# Autodesk Inventor assembly: Assembly1
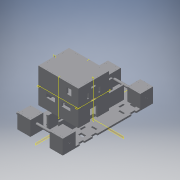
[picture p0: Inventor's stored thumbnail of the model, 180x180]
Saved by Autodesk Inventor 2019 (Build 230136000, 136)
## iProperties
Created: 2018-05-14
Part Number: Assembly1
Document SubType Name: Assembly
Designer: Administrator
Author: Administrator
## Documents named in this file (16)
- E:\New folder\Assembly1.iam
- E:\New folder\Part1.ipt
- E:\New folder\Part2.ipt
- E:\New folder\Part3.ipt
- E:\New folder\Part4.ipt
- E:\New folder\Part5.ipt
- E:\New folder\Part6.ipt
- E:\New folder\Part7.ipt
- E:\New folder\Part8.ipt
- E:\New folder\Part9.ipt
- E:\New folder\Part10.ipt
- E:\New folder\Part11.ipt
- E:\New folder\Part12.ipt
- E:\New folder\Part13.ipt
- E:\New folder\Part14.ipt
- E:\New folder\Part15.ipt
## Components (36 placed, 15 different names)
1. Part1:1 — Flush:49, Flush:50, Flush:51, Flush:52, Flush:53, Flush:54, Flush:55, Flush:56, Flush:57, Flush:58, Flush:59, Flush:60, Flush:61, Mate:1, Mate:2, Mate:3, Mate:4, Flush:62, Mate:5, Mate:6, Mate:7, Mate:8, Flush:79, Mate:14
2. Part2:1 — Flush:1, Flush:2, Flush:3, Flush:9, Flush:10, Flush:60, Insert:2
3. Part2:2 — Flush:4, Flush:5, Flush:6, Flush:7, Flush:8
4. Part3:1 — Flush:1, Flush:2, Flush:3, Flush:4, Flush:5, Flush:6, Flush:11, Flush:12
5. Part3:2 — Flush:7, Flush:8, Flush:9, Flush:56, Flush:57
6. Part4:1 — Flush:10, Flush:11, Flush:12
7. Part2:3
8. Part2:4 — Flush:59
9. Part3:3
10. Part3:4 — Flush:55, Flush:58
11. Part4:2
12. Part2:5 — Flush:54, Insert:1
13. Part2:6 — Flush:52
14. Part3:5 — Flush:53
15. Part3:6
16. Part4:3
17. Part2:7 — Flush:51
18. Part2:8 — Flush:50
19. Part3:7 — Flush:49
20. Part3:8
21. Part4:4
22. Part5:1 — Flush:61, Mate:1, Mate:2
23. Part5:2 — Mate:3, Mate:4, Flush:62
24. Part6:1 — Insert:2
25. Part6:2 — Insert:1
26. Part7:1 — Mate:5, Mate:6, Mate:7
27. Part8:1 — Flush:69, Flush:70, Flush:71, Flush:76, Flush:77, Mate:8
28. Part9:1 — Flush:66, Flush:67, Flush:68, Flush:72, Flush:75
29. Part10:1 — Flush:63, Flush:64, Flush:65, Flush:66, Flush:67, Flush:68, Flush:73, Flush:74
30. Part11:1 — Flush:63, Flush:64, Flush:65, Flush:69, Flush:70, Flush:71
31. Part12:1 — Flush:75, Flush:76, Flush:77, Flush:79, Flush:86, Mate:12, Mate:13
32. Part13:1 — Flush:72, Flush:73, Flush:74
33. Part14:1 — Flush:80, Flush:81, Mate:9, Mate:11, Flush:84, Flush:85
34. Part15:1 — Flush:80, Flush:81, Mate:9, Flush:86, Mate:12, Mate:13
35. Part14:2
36. Part15:2 — Mate:11, Flush:84, Flush:85, Mate:14
## Relationships (101: Flush 85, Mate 14, Insert 2)
- Flush:1: Part2:1 ↔ Part3:1
- Flush:2: Part2:1 ↔ Part3:1
- Flush:3: Part2:1 ↔ Part3:1
- Flush:4: Part2:2 ↔ Part3:1
- Flush:5: Part2:2 ↔ Part3:1
- Flush:6: Part2:2 ↔ Part3:1
- Flush:7: Part2:2 ↔ Part3:2
- Flush:8: Part2:2 ↔ Part3:2
- Flush:9: Part2:1 ↔ Part3:2
- Flush:10: Part2:1 ↔ Part4:1
- Flush:11: Part3:1 ↔ Part4:1
- Flush:12: Part3:1 ↔ Part4:1
- [Flush]: Part2:3 ↔ Part3:3
- [Flush]: Part2:3 ↔ Part3:3
- [Flush]: Part2:3 ↔ Part3:3
- [Flush]: Part2:4 ↔ Part3:3
- [Flush]: Part2:4 ↔ Part3:3
- [Flush]: Part2:4 ↔ Part3:3
- [Flush]: Part2:4 ↔ Part3:4
- [Flush]: Part2:4 ↔ Part3:4
- [Flush]: Part2:3 ↔ Part3:4
- [Flush]: Part2:3 ↔ Part4:2
- [Flush]: Part3:3 ↔ Part4:2
- [Flush]: Part3:3 ↔ Part4:2
- [Flush]: Part2:5 ↔ Part3:5
- [Flush]: Part2:5 ↔ Part3:5
- [Flush]: Part2:5 ↔ Part3:5
- [Flush]: Part2:6 ↔ Part3:5
- [Flush]: Part2:6 ↔ Part3:5
- [Flush]: Part2:6 ↔ Part3:5
- [Flush]: Part2:6 ↔ Part3:6
- [Flush]: Part2:6 ↔ Part3:6
- [Flush]: Part2:5 ↔ Part3:6
- [Flush]: Part2:5 ↔ Part4:3
- [Flush]: Part3:5 ↔ Part4:3
- [Flush]: Part3:5 ↔ Part4:3
- [Flush]: Part2:7 ↔ Part3:7
- [Flush]: Part2:7 ↔ Part3:7
- [Flush]: Part2:7 ↔ Part3:7
- [Flush]: Part2:8 ↔ Part3:7
- [Flush]: Part2:8 ↔ Part3:7
- [Flush]: Part2:8 ↔ Part3:7
- [Flush]: Part2:8 ↔ Part3:8
- [Flush]: Part2:8 ↔ Part3:8
- [Flush]: Part2:7 ↔ Part3:8
- [Flush]: Part2:7 ↔ Part4:4
- [Flush]: Part3:7 ↔ Part4:4
- [Flush]: Part3:7 ↔ Part4:4
- Flush:49: Part1:1 ↔ Part3:7
- Flush:50: Part1:1 ↔ Part2:8
- Flush:51: Part1:1 ↔ Part2:7
- Flush:52: Part1:1 ↔ Part2:6
- Flush:53: Part1:1 ↔ Part3:5
- Flush:54: Part1:1 ↔ Part2:5
- Flush:55: Part1:1 ↔ Part3:4
- Flush:56: Part1:1 ↔ Part3:2
- Flush:57: Part1:1 ↔ Part3:2
- Flush:58: Part1:1 ↔ Part3:4
- Flush:59: Part1:1 ↔ Part2:4
- Flush:60: Part1:1 ↔ Part2:1
- Flush:61: Part1:1 ↔ Part5:1
- Mate:1: Part1:1 ↔ Part5:1
- Mate:2: Part1:1 ↔ Part5:1
- Mate:3: Part1:1 ↔ Part5:2
- Mate:4: Part1:1 ↔ Part5:2
- Flush:62: Part1:1 ↔ Part5:2
- Insert:1: Part2:5 ↔ Part6:2
- Insert:2: Part2:1 ↔ Part6:1
- Mate:5: Part1:1 ↔ Part7:1
- Mate:6: Part1:1 ↔ Part7:1
- Mate:7: Part1:1 ↔ Part7:1
- Flush:63: Part10:1 ↔ Part11:1
- Flush:64: Part10:1 ↔ Part11:1
- Flush:65: Part10:1 ↔ Part11:1
- Flush:66: Part9:1 ↔ Part10:1
- Flush:67: Part9:1 ↔ Part10:1
- Flush:68: Part9:1 ↔ Part10:1
- Flush:69: Part8:1 ↔ Part11:1
- Flush:70: Part8:1 ↔ Part11:1
- Flush:71: Part8:1 ↔ Part11:1
- Flush:72: Part9:1 ↔ Part13:1
- Flush:73: Part10:1 ↔ Part13:1
- Flush:74: Part10:1 ↔ Part13:1
- Flush:75: Part9:1 ↔ Part12:1
- Flush:76: Part8:1 ↔ Part12:1
- Flush:77: Part8:1 ↔ Part12:1
- Mate:8 (25.4 mm): Part1:1 ↔ Part8:1
- Flush:79 (7.62 mm): Part1:1 ↔ Part12:1
- Flush:80: Part14:1 ↔ Part15:1
- Flush:81: Part14:1 ↔ Part15:1
- Mate:9: Part14:1 ↔ Part15:1
- [Flush]: Part14:2 ↔ Part15:2
- [Flush]: Part14:2 ↔ Part15:2
- [Mate]: Part14:2 ↔ Part15:2
- Mate:11: Part14:1 ↔ Part15:2
- Flush:84: Part14:1 ↔ Part15:2
- Flush:85: Part14:1 ↔ Part15:2
- Flush:86: Part12:1 ↔ Part15:1
- Mate:12: Part12:1 ↔ Part15:1
- Mate:13: Part12:1 ↔ Part15:1
- Mate:14: Part1:1 ↔ Part15:2
## Named parameters: d12_d1 = 0 mm, d13_d2 = 0 mm, d14_d3 = 0 mm, d15_d4 = 0 mm, d16_d5 = 0 mm, d17_d6 = 0 mm, d18_d7 = 0 mm, d19_d8 = 0 mm, d20_d9 = 0 mm, d21_d10 = 0 mm, d22_d11 = 0 mm, d23_d0 = 0 mm, d24_d1 = 0 mm, d25_d2 = 0 mm, d26_d3 = 0 mm, d27_d4 = 0 mm, d28_d5 = 0 mm, d29_d6 = 0 mm, d30_d7 = 0 mm, d31_d8 = 0 mm, d32_d9 = 0 mm, d33_d10 = 0 mm, d34_d11 = 0 mm, d35_d0 = 0 mm, d36_d1 = 0 mm, d37_d2 = 0 mm, d38_d3 = 0 mm, d39_d4 = 0 mm, d40_d5 = 0 mm, d41_d6 = 0 mm, d42_d7 = 0 mm, d43_d8 = 0 mm, d44_d9 = 0 mm, d45_d10 = 0 mm, d46_d11 = 0 mm, d47_d0 = 0 mm, d94_d93 = 0 mm, d95_d91 = 0 mm, d96_d92 = 0 mm
